# Autodesk Inventor assembly: PolarizationMethod
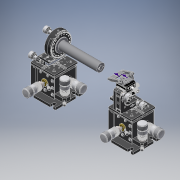
[picture p0: Inventor's stored thumbnail of the model, 180x180]
Saved by Autodesk Inventor 2019 (Build 230136000, 136)
## iProperties
Created: 2019-05-24
Part Number: PolarizationMethod
Document SubType Name: Assembly
Designer: aorfi
Author: aorfi
## Documents named in this file (10)
- C:\Users\aorfi\Documents\IQC\PolarizationMethod.iam
- C:\Users\aorfi\Documents\IQC\COTS\ThorLabs\3AxisStage-MBT616D.ipt
- C:\Users\aorfi\Documents\IQC\COTS\ThorLabs\RollStage-RSP1_M.ipt
- C:\Users\aorfi\Documents\IQC\COTS\ThorLabs\YawPitchStage-KM100PM.ipt
- C:\Users\aorfi\Documents\IQC\ChipMountAssembly.iam
- C:\Users\aorfi\Documents\IQC\CustomParts\FiberMount.ipt
- C:\Users\aorfi\Documents\IQC\CustomParts\EpoxyFiberMountBase.ipt
- C:\Users\aorfi\Documents\IQC\CustomParts\FixedFiber.ipt
- C:\Users\aorfi\Documents\IQC\CustomParts\RubayetChip.ipt
- C:\Users\aorfi\Documents\IQC\COTS\ThorLabs\2StageDoveTail-DT12XY.ipt
## Components (12 placed, 9 different names)
1. 3AxisStage-MBT616D:1 — Mate:1, Flush:1, Mate:2, Flush:3, Flush:5
2. 3AxisStage-MBT616D:2 — Mate:6, Flush:4, Flush:5, Mate:8, Mate:12, Flush:7
3. RollStage-RSP1_M:1 — Mate:4, Angle:1, Mate:5, Mate:7, Mate:13, Mate:14
4. YawPitchStage-KM100PM:1 — Mate:2, Mate:4, Angle:1, Mate:13
5. ChipMountAssembly:1 [sub-assembly] — Mate:5, Mate:7
6. YawPitchStage-KM100PM:2 — Mate:8, Mate:12, Flush:7, Mate:27, Flush:11
7. FiberMount:1 — Mate:24, Mate:25, Mate:26, Flush:10, Mate:30
8. EpoxyFiberMountBase:1 — Mate:24, Mate:29, Mate:30, Flush:12, Mate:31
9. FixedFiber:1 — Mate:22, Mate:23, Flush:8
10. RubayetChip:1 — Mate:22, Mate:23, Flush:8
11. RubayetChip:2 — Mate:25, Mate:26, Flush:10
12. 2StageDoveTail-DT12XY:1 — Mate:27, Flush:11, Mate:28, Mate:29, Mate:31
## Relationships (30: Mate 20, Flush 9, Angle 1)
- Mate:1: 3AxisStage-MBT616D:1
- Flush:1: 3AxisStage-MBT616D:1
- Mate:2: 3AxisStage-MBT616D:1 ↔ YawPitchStage-KM100PM:1
- Mate:4: RollStage-RSP1_M:1 ↔ YawPitchStage-KM100PM:1
- Flush:3: 3AxisStage-MBT616D:1
- Angle:1 (180 deg): RollStage-RSP1_M:1 ↔ YawPitchStage-KM100PM:1
- Mate:5: RollStage-RSP1_M:1 ↔ ChipMountAssembly:1
- Mate:6: 3AxisStage-MBT616D:2
- Flush:4: 3AxisStage-MBT616D:2
- Flush:5 (-200 mm): 3AxisStage-MBT616D:1 ↔ 3AxisStage-MBT616D:2
- Mate:7: RollStage-RSP1_M:1 ↔ ChipMountAssembly:1
- Mate:8: 3AxisStage-MBT616D:2 ↔ YawPitchStage-KM100PM:2
- Mate:12 (5 mm): 3AxisStage-MBT616D:2 ↔ YawPitchStage-KM100PM:2
- Flush:7: 3AxisStage-MBT616D:2 ↔ YawPitchStage-KM100PM:2
- Mate:13: RollStage-RSP1_M:1 ↔ YawPitchStage-KM100PM:1
- Mate:14: RollStage-RSP1_M:1
- Mate:22: FixedFiber:1 ↔ RubayetChip:1
- Mate:23: FixedFiber:1 ↔ RubayetChip:1
- Flush:8: FixedFiber:1 ↔ RubayetChip:1
- Mate:24: FiberMount:1 ↔ EpoxyFiberMountBase:1
- Mate:25: FiberMount:1 ↔ RubayetChip:2
- Mate:26: FiberMount:1 ↔ RubayetChip:2
- Flush:10: FiberMount:1 ↔ RubayetChip:2
- Mate:27: YawPitchStage-KM100PM:2 ↔ 2StageDoveTail-DT12XY:1
- Flush:11 (-3 mm): YawPitchStage-KM100PM:2 ↔ 2StageDoveTail-DT12XY:1
- Mate:28: 2StageDoveTail-DT12XY:1
- Mate:29: EpoxyFiberMountBase:1 ↔ 2StageDoveTail-DT12XY:1
- Mate:30: FiberMount:1 ↔ EpoxyFiberMountBase:1
- Flush:12: EpoxyFiberMountBase:1
- Mate:31: EpoxyFiberMountBase:1 ↔ 2StageDoveTail-DT12XY:1
